# Autodesk Inventor assembly: IMX178 Camera Case Assembly
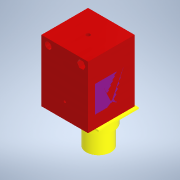
[picture p0: Inventor's stored thumbnail of the model, 180x180]
Saved by Autodesk Inventor 2022.1 (Build 261234000, 234)
## iProperties
Created: 2021-07-25
Part Number: IMX178 Camera Case Assembly
Document SubType Name: Assembly
Designer: robst
Author: robst
## Documents named in this file (6)
- C:\git\CAD-Development\robSteele\ShapeWays\GlobalMeteorNetwork\IMX178 Camera Case Assembly.iam
- C:\git\CAD-Development\robSteele\ShapeWays\GlobalMeteorNetwork\IMX178 Camera Case Telescope Attachement.ipt
- C:\git\CAD-Development\robSteele\ShapeWays\GlobalMeteorNetwork\IMX178 Camera Case Bottom.ipt
- C:\git\CAD-Development\robSteele\ShapeWays\GlobalMeteorNetwork\IMX178 Camera Case.ipt
- C:\git\CAD-Development\robSteele\ShapeWays\GlobalMeteorNetwork\IMX178 Camera Case Cap.ipt
- C:\git\CAD-Development\robSteele\ShapeWays\GlobalMeteorNetwork\IMX178 Shell For Ethernet Strain Relief.ipt
## Components (5 placed, 5 different names)
1. IMX178 Camera Case:1 — Mate:1, Flush:1, Flush:2, Mate:2, Flush:3, Flush:4
2. IMX178 Camera Case Telescope Attachement:1 — Mate:3, Flush:5, Flush:6
3. IMX178 Camera Case Bottom:1 — Mate:1, Flush:1, Flush:2, Mate:4
4. IMX178 Camera Case Cap:1 — Mate:2, Flush:3, Flush:4, Mate:3, Flush:5, Flush:6, Flush:7, Flush:8
5. IMX178 Shell For Ethernet Strain Relief:1 — Mate:4, Flush:7, Flush:8
## Relationships (12: Flush 8, Mate 4)
- Mate:1: IMX178 Camera Case:1 ↔ IMX178 Camera Case Bottom:1
- Flush:1: IMX178 Camera Case:1 ↔ IMX178 Camera Case Bottom:1
- Flush:2: IMX178 Camera Case:1 ↔ IMX178 Camera Case Bottom:1
- Mate:2: IMX178 Camera Case:1 ↔ IMX178 Camera Case Cap:1
- Flush:3: IMX178 Camera Case:1 ↔ IMX178 Camera Case Cap:1
- Flush:4: IMX178 Camera Case:1 ↔ IMX178 Camera Case Cap:1
- Mate:3: IMX178 Camera Case Telescope Attachement:1 ↔ IMX178 Camera Case Cap:1
- Flush:5: IMX178 Camera Case Telescope Attachement:1 ↔ IMX178 Camera Case Cap:1
- Flush:6: IMX178 Camera Case Telescope Attachement:1 ↔ IMX178 Camera Case Cap:1
- Mate:4: IMX178 Camera Case Bottom:1 ↔ IMX178 Shell For Ethernet Strain Relief:1
- Flush:7: IMX178 Camera Case Cap:1 ↔ IMX178 Shell For Ethernet Strain Relief:1
- Flush:8: IMX178 Camera Case Cap:1 ↔ IMX178 Shell For Ethernet Strain Relief:1
